# Autodesk Inventor assembly: アームアセンブリ
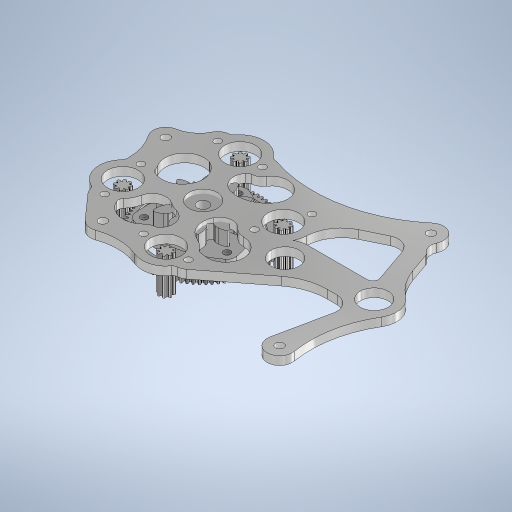
[picture p0: Inventor's stored thumbnail of the model, 512x512]
Saved by Autodesk Inventor 2023 (Build 270158000, 158)
## iProperties
Created: 2022-03-06
Part Number: アームアセンブリ
Document SubType Name: Assembly
Designer: acps
Author: acps
## Documents named in this file (4)
- C:\Users\acps\Documents\srdc\srdc_ksh\アーム\アームアセンブリ.iam
- C:\Users\acps\Documents\srdc\srdc_ksh\アーム\モータマウント.ipt
- C:\Users\acps\Documents\srdc\srdc_ksh\アーム\ギア\ぴにょんz8.ipt
- C:\Users\acps\Documents\srdc\srdc_ksh\アーム\ギア\初段_多段ギア.iam
## Components (6 placed, 3 different names)
1. モータマウント:1 — Mate:1, Mate:2, Mate:3, Mate:4, Mate:5
2. ぴにょんz8:1 — Mate:1
3. ぴにょんz8:2 — Mate:2
4. ぴにょんz8:3 — Mate:3
5. ぴにょんz8:4 — Mate:4
6. 初段_多段ギア:1 [sub-assembly] — Mate:5
## Relationships (5: Mate 5)
- Mate:1: モータマウント:1 ↔ ぴにょんz8:1
- Mate:2: モータマウント:1 ↔ ぴにょんz8:2
- Mate:3: モータマウント:1 ↔ ぴにょんz8:3
- Mate:4: モータマウント:1 ↔ ぴにょんz8:4
- Mate:5: モータマウント:1 ↔ 初段_多段ギア:1
